# Autodesk Inventor assembly: arduino_with_case
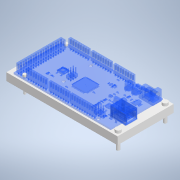
[picture p0: Inventor's stored thumbnail of the model, 180x180]
Saved by Autodesk Inventor 2021.4 (Build 254397000, 397)
## iProperties
Created: 2022-07-26
Part Number: arduino_with_case
Document SubType Name: Assembly
Designer: isamu
Author: isamu
## Documents named in this file (5)
- D:\personal_projects\robot\inventor\2021_matlab_compat _v2\servo_frames\arduino_with_case.iam
- D:\personal_projects\robot\exports\arduino_mega_case.ipt
- D:\personal_projects\robot\exports\arduino_mega.ipt
- D:\personal_projects\robot\exports\screws\m3x16.ipt
- D:\personal_projects\robot\exports\screws\m2x16.ipt
## Components (6 placed, 4 different names)
1. arduino_mega_case:1 — Mate:1, Mate:2, Mate:3, Insert:1, Insert:2
2. arduino_mega:1 — Mate:1, Mate:2, Mate:3, Insert:3, Insert:4
3. m3x16:1 — Insert:1
4. m3x16:2 — Insert:2
5. m2x16:1 — Insert:3
6. m2x16:2 — Insert:4
## Relationships (7: Insert 4, Mate 3)
- Mate:1: arduino_mega_case:1 ↔ arduino_mega:1
- Mate:2: arduino_mega_case:1 ↔ arduino_mega:1
- Mate:3: arduino_mega_case:1 ↔ arduino_mega:1
- Insert:1: arduino_mega_case:1 ↔ m3x16:1
- Insert:2: arduino_mega_case:1 ↔ m3x16:2
- Insert:3: arduino_mega:1 ↔ m2x16:1
- Insert:4: arduino_mega:1 ↔ m2x16:2
